# Autodesk Inventor assembly: 0401 ASY GBK wall shield Center 1
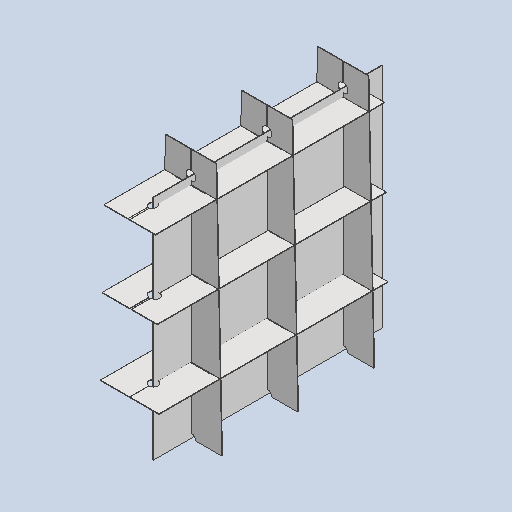
[picture p0: Inventor's stored thumbnail of the model, 512x512]
Saved by Autodesk Inventor 2026.2 (Build 302298000, 298)
## iProperties
Created: 2026-05-19
Part Number: 0401 ASY GBK wall shield Center 1
Document SubType Name: Assembly
Designer: admin
Mass: 174041 g
Surface Area: 113034 cm^2
Volume: 22170.8 cm^3
Density: 7.85 g/cm^3
Author: admin
## Documents named in this file (6)
- C:\Users\admin\Documents\Inventor\GBK-Gubkinskiy\0401 ASY GBK wall shield Center 1.iam
- C:\Users\admin\Documents\Inventor\GBK-Gubkinskiy\0411 GBK Center main rib.ipt
- C:\Users\admin\Documents\Inventor\GBK-Gubkinskiy\0413 GBK stringer C1.ipt
- C:\Users\admin\Documents\Inventor\GBK-Gubkinskiy\01.1 GBK shield.ipt
- C:\Users\admin\Documents\Inventor\GBK-Gubkinskiy\0414 GBK stringer C2.ipt
- C:\Users\admin\Documents\Inventor\GBK-Gubkinskiy\0415 GBK stringer C3.ipt
## Components (13 placed, 5 different names)
1. 0413 GBK stringer C1:1 — Rigid:1
2. Part111:1 — Mate:1, Flush:1, Mate:2, Flush:2, Mate:4, Flush:3, Mate:5, Flush:5
3. 0414 GBK stringer C2:1 — Rigid:2
4. 0415 GBK stringer C3:1 — Rigid:3
5. 0413 GBK stringer C1:2 — Rigid:6
6. 0414 GBK stringer C2:2 — Rigid:5
7. 0415 GBK stringer C3:2 — Rigid:4
8. 0411 GBK Center main rib:1 — Rigid:1, Flush:3, Mate:5, Flush:4, Flush:5, Rigid:2, Rigid:3
9. 0411 GBK Center main rib:2 — Flush:2, Mate:4, Flush:4, Rigid:4, Rigid:5, Rigid:6
10. 0411 GBK Center main rib:3
11. 0411 GBK Center main rib:4
12. 0411 GBK Center main rib:5
13. 0411 GBK Center main rib:6
## Component patterns: (3 elements, first: 0411 GBK Center main rib:1 + 0411 GBK Center main rib:2)
## Relationships (15: WeldJoint 6, Flush 5, Mate 4)
- Rigid:1 [WeldJoint] (4 mm): 0413 GBK stringer C1:1 ↔ 0411 GBK Center main rib:1
- Mate:1: Part111:1
- Flush:1: Part111:1
- Mate:2: Part111:1
- Flush:2: Part111:1 ↔ 0411 GBK Center main rib:2
- Mate:4: Part111:1 ↔ 0411 GBK Center main rib:2
- Flush:3: Part111:1 ↔ 0411 GBK Center main rib:1
- Mate:5: Part111:1 ↔ 0411 GBK Center main rib:1
- Flush:4: 0411 GBK Center main rib:1 ↔ 0411 GBK Center main rib:2
- Flush:5 (250 mm): Part111:1 ↔ 0411 GBK Center main rib:1
- Rigid:2 [WeldJoint] (4 mm): 0414 GBK stringer C2:1 ↔ 0411 GBK Center main rib:1
- Rigid:3 [WeldJoint] (4 mm): 0415 GBK stringer C3:1 ↔ 0411 GBK Center main rib:1
- Rigid:4 [WeldJoint]: 0415 GBK stringer C3:2 ↔ 0411 GBK Center main rib:2
- Rigid:5 [WeldJoint]: 0414 GBK stringer C2:2 ↔ 0411 GBK Center main rib:2
- Rigid:6 [WeldJoint]: 0413 GBK stringer C1:2 ↔ 0411 GBK Center main rib:2
